# Autodesk Inventor assembly: SM-XZA1
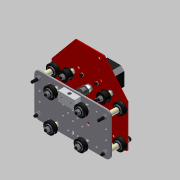
[picture p0: Inventor's stored thumbnail of the model, 180x180]
Saved by Autodesk Inventor 2012 SP1 (Build 160190100, 190)
## iProperties
Created: 2012-05-01
Part Number: SM-XZA1
Document SubType Name: Assembly
Designer: ERF
Stock Number: SM-XZA1
Author: ERF
Title: X/Z Carriage Assembly
## Documents named in this file (3)
- C:\Users\eford\Documents\Projects\Shapoko_v1i\Workspaces\Workspace\Projects\USER FOLDER\Edward\Shapeoko_v1i\Assemblies\SM-XZA1.iam
- C:\Users\eford\Documents\Projects\Shapoko_v1i\Workspaces\Workspace\Projects\USER FOLDER\Edward\Shapeoko_v1i\Assemblies\SM-ZA01.iam
- C:\Users\eford\Documents\Projects\Shapoko_v1i\Workspaces\Workspace\Projects\USER FOLDER\Edward\Shapeoko_v1i\Assemblies\SM-XA01.iam
## Components (2 placed, 2 different names)
1. SM-ZA01:1 [sub-assembly] — Insert:1, Insert:2
2. SM-XA01:1 [sub-assembly] — Insert:1, Insert:2
## Relationships (2: Insert 2)
- Insert:1: SM-ZA01:1 ↔ SM-XA01:1
- Insert:2: SM-ZA01:1 ↔ SM-XA01:1
